# Autodesk Inventor assembly: Assembly
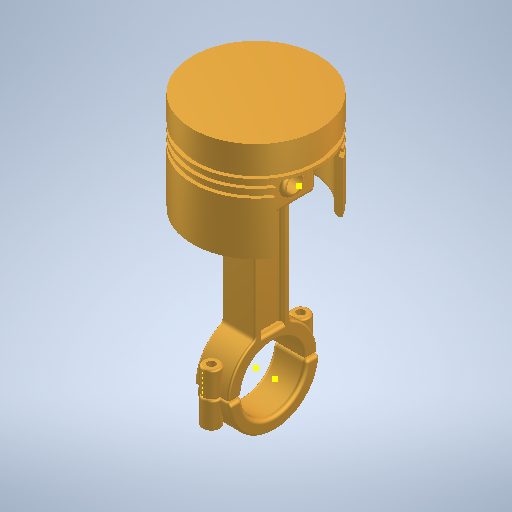
[picture p0: Inventor's stored thumbnail of the model, 512x512]
Saved by Autodesk Inventor 2025.1 (Build 291241000, 241)
## iProperties
Created: 2024-08-01
Part Number: Assembly
Document SubType Name: Assembly
Designer: vedan
Author: vedan
## Documents named in this file (5)
- C:\Users\vedan\OneDrive\Desktop\CAD\assemblies\EnginePiston\Assembly.iam
- C:\Users\vedan\OneDrive\Desktop\CAD\assemblies\EnginePiston\PistonHead.ipt
- C:\Users\vedan\OneDrive\Desktop\CAD\assemblies\EnginePiston\PistonPin.ipt
- C:\Users\vedan\OneDrive\Desktop\CAD\assemblies\EnginePiston\PistonRod.ipt
- C:\Users\vedan\OneDrive\Desktop\CAD\assemblies\EnginePiston\PistonRodCap.ipt
## Components (4 placed, 4 different names)
1. PistonHead:1 — Mate:1, Mate:2, Mate:3
2. PistonPin:1 — Mate:2, Mate:3
3. PistonRod:1 — Mate:1, Mate:4
4. PistonRodCap:1 — Mate:4
## Relationships (4: Mate 4)
- Mate:1: PistonHead:1 ↔ PistonRod:1
- Mate:2: PistonHead:1 ↔ PistonPin:1
- Mate:3: PistonHead:1 ↔ PistonPin:1
- Mate:4: PistonRod:1 ↔ PistonRodCap:1
